# Autodesk Inventor assembly: segment0
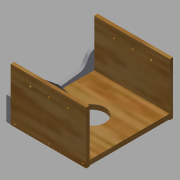
[picture p0: Inventor's stored thumbnail of the model, 180x180]
Saved by Autodesk Inventor 2013 (Build 170138000, 138)
## iProperties
Created: 2014-10-10
Part Number: segment0
Document SubType Name: Assembly
Designer: Masta
Author: Masta
## Documents named in this file (5)
- D:\DrOctopus\3D model\arm\segment0.iam
- D:\DrOctopus\3D model\arm\servo arm TGY-S8166M double.ipt
- D:\DrOctopus\3D model\arm\segment0a.ipt
- D:\DrOctopus\3D model\arm\segment0b.ipt
- D:\DrOctopus\3D model\arm\segment0c.ipt
## Components (5 placed, 4 different names)
1. servo arm TGY-S8166M double:1 — Insert:1, Insert:2
2. segment0a:1 — Mate:1, Flush:2, Flush:3, Insert:1, Insert:2
3. segment0a:2 — Mate:2, Flush:4, Flush:5
4. segment0b:1 — Mate:1, Flush:2, Flush:3, Mate:2, Flush:4, Flush:5, Flush:6
5. segment0c:1 — Flush:6
## Relationships (9: Flush 5, Mate 2, Insert 2)
- Mate:1: segment0a:1 ↔ segment0b:1
- Flush:2: segment0a:1 ↔ segment0b:1
- Flush:3: segment0a:1 ↔ segment0b:1
- Mate:2: segment0a:2 ↔ segment0b:1
- Flush:4: segment0a:2 ↔ segment0b:1
- Flush:5: segment0a:2 ↔ segment0b:1
- Insert:1: servo arm TGY-S8166M double:1 ↔ segment0a:1
- Insert:2: servo arm TGY-S8166M double:1 ↔ segment0a:1
- Flush:6: segment0b:1 ↔ segment0c:1
